# Autodesk Inventor assembly: Assembly1
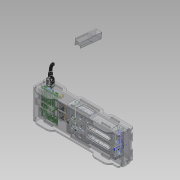
[picture p0: Inventor's stored thumbnail of the model, 180x180]
Saved by Autodesk Inventor 2016 (Build 200138000, 138)
## iProperties
Created: 2015-06-16
Part Number: Assembly1
Document SubType Name: Assembly
Designer: Openlab
Author: Openlab
## Documents named in this file (12)
- E:\Alex\DI-Lambda\parts\Paris\Assembly.iam
- E:\Alex\DI-Lambda\parts\Paris\LED_board.ipt
- E:\Alex\DI-Lambda\parts\Paris\Sensor_board.ipt
- E:\Alex\DI-Lambda\parts\Paris\Box_top.ipt
- E:\Alex\DI-Lambda\parts\Paris\Box_bottom.ipt
- E:\Alex\DI-Lambda\parts\Paris\Box_left_wall.ipt
- E:\Alex\DI-Lambda\parts\Paris\Microcontroller_board_Paris.iam
- E:\Alex\DI-Lambda\parts\Paris\Box_back_wall.ipt
- E:\Alex\DI-Lambda\parts\Paris\Box_front_wall.ipt
- E:\Alex\DI-Lambda\parts\Common\Cuvette.ipt
- E:\Alex\DI-Lambda\parts\Paris\Core_bottom-im.ipt
- E:\Alex\DI-Lambda\parts\Paris\Core_top-im.ipt
## Components (12 placed, 11 different names)
1. LED_board:1 — Mate:95, Mate:96, Mate:97
2. Sensor_board:1 — Mate:98, Mate:99, Mate:100
3. Box_top:1 — Mate:76, Mate:77, Mate:78, Mate:84, Mate:86, Mate:92, Mate:103, Mate:104
4. Box_bottom:1 — Mate:79, Mate:80, Mate:81, Mate:102
5. Box_left_wall:1 — Mate:83, Mate:84, Mate:85, Mate:91
6. Microcontroller_board_Paris:1 [sub-assembly] — Mate:89, Mate:90, Mate:91
7. Box_back_wall:1 — Mate:76, Mate:77, Mate:78, Mate:79, Mate:80, Mate:81, Mate:83, Mate:85, Mate:87, Mate:88
8. Box_front_wall:1 — Mate:92, Mate:93, Mate:94
9. Box_left_wall:2 — Mate:86, Mate:87, Mate:88, Mate:89, Mate:90, Mate:93, Mate:94
10. Cuvette:1
11. Core_bottom-im:1 — Mate:95, Mate:96, Mate:97, Mate:98, Mate:99, Mate:100, Mate:101, Flush:1, Flush:2, Mate:102
12. Core_top-im:1 — Mate:101, Flush:1, Flush:2, Mate:103, Mate:104
## Relationships (30: Mate 28, Flush 2)
- Mate:76: Box_top:1 ↔ Box_back_wall:1
- Mate:77: Box_top:1 ↔ Box_back_wall:1
- Mate:78: Box_top:1 ↔ Box_back_wall:1
- Mate:79: Box_bottom:1 ↔ Box_back_wall:1
- Mate:80: Box_bottom:1 ↔ Box_back_wall:1
- Mate:81: Box_bottom:1 ↔ Box_back_wall:1
- Mate:83: Box_left_wall:1 ↔ Box_back_wall:1
- Mate:84: Box_top:1 ↔ Box_left_wall:1
- Mate:85: Box_left_wall:1 ↔ Box_back_wall:1
- Mate:86: Box_top:1 ↔ Box_left_wall:2
- Mate:87: Box_back_wall:1 ↔ Box_left_wall:2
- Mate:88: Box_back_wall:1 ↔ Box_left_wall:2
- Mate:89: Microcontroller_board_Paris:1 ↔ Box_left_wall:2
- Mate:90: Microcontroller_board_Paris:1 ↔ Box_left_wall:2
- Mate:91: Box_left_wall:1 ↔ Microcontroller_board_Paris:1
- Mate:92: Box_top:1 ↔ Box_front_wall:1
- Mate:93: Box_front_wall:1 ↔ Box_left_wall:2
- Mate:94: Box_front_wall:1 ↔ Box_left_wall:2
- Mate:95: LED_board:1 ↔ Core_bottom-im:1
- Mate:96 (0.5 mm): LED_board:1 ↔ Core_bottom-im:1
- Mate:97: LED_board:1 ↔ Core_bottom-im:1
- Mate:98: Sensor_board:1 ↔ Core_bottom-im:1
- Mate:99 (0.5 mm): Sensor_board:1 ↔ Core_bottom-im:1
- Mate:100: Sensor_board:1 ↔ Core_bottom-im:1
- Mate:101: Core_bottom-im:1 ↔ Core_top-im:1
- Flush:1: Core_bottom-im:1 ↔ Core_top-im:1
- Flush:2: Core_bottom-im:1 ↔ Core_top-im:1
- Mate:102: Box_bottom:1 ↔ Core_bottom-im:1
- Mate:103: Box_top:1 ↔ Core_top-im:1
- Mate:104: Box_top:1 ↔ Core_top-im:1
